# Autodesk Inventor assembly: 240531_3Dstorage1
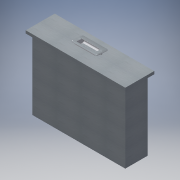
[picture p0: Inventor's stored thumbnail of the model, 180x180]
Saved by Autodesk Inventor 2016 (Build 200138000, 138)
## iProperties
Created: 2024-05-31
Part Number: 240531_3Dstorage1
Material: 일반
Document SubType Name: Assembly
Designer: pc
Author: pc
## Documents named in this file (3)
- D:\CAD_HCH\240531\240531_3Dstorage1.iam
- D:\CAD_HCH\240531\240531_3Dstorage2.ipt
- D:\CAD_HCH\240531\240531_3Dstorage3.ipt
## Components (2 placed, 2 different names)
1. 240531_3Dstorage2:1 — 메이트:1
2. 240531_3Dstorage3:1 — 메이트:1
## Relationships (1: Mate 1)
- 메이트:1 [Mate]: 240531_3Dstorage2:1 ↔ 240531_3Dstorage3:1
